# Autodesk Inventor assembly: nozzle
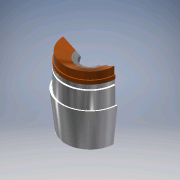
[picture p0: Inventor's stored thumbnail of the model, 180x180]
Saved by Autodesk Inventor 2017 (Build 210142000, 142)
## iProperties
Created: 2016-10-21
Part Number: nozzle
Document SubType Name: Assembly
Designer: cmflanne
Author: cmflanne
## Documents named in this file (7)
- C:\Users\cmflanne\Downloads\Intrepid\Nozzle\nozzle.iam
- C:\Users\cmflanne\Downloads\Intrepid\Nozzle\aluminum_carrier.ipt
- C:\Users\cmflanne\Downloads\Intrepid\Nozzle\aluminum_retainer.ipt
- C:\Users\cmflanne\Downloads\Intrepid\Nozzle\aluminum_skirt.ipt
- C:\Users\cmflanne\Downloads\Intrepid\Nozzle\graphite.ipt
- C:\Users\cmflanne\Downloads\Intrepid\Nozzle\phenolic_cap.ipt
- C:\Users\cmflanne\Downloads\Intrepid\Nozzle\phenolic_carrier.ipt
## Components (6 placed, 6 different names)
1. aluminum_carrier:1 — Mate:5, Mate:8, Mate:9, Mate:10
2. aluminum_retainer:1 — Mate:4, Mate:9
3. aluminum_skirt:1 — Mate:3, Mate:10
4. graphite:1 — Mate:1, Mate:2, Mate:3, Mate:4, Mate:5, Mate:6, Mate:7
5. phenolic_cap:1 — Mate:1, Mate:6, Mate:8
6. phenolic_carrier:1 — Mate:2, Mate:7
## Relationships (10: Mate 10)
- Mate:1: graphite:1 ↔ phenolic_cap:1
- Mate:2: graphite:1 ↔ phenolic_carrier:1
- Mate:3: aluminum_skirt:1 ↔ graphite:1
- Mate:4: aluminum_retainer:1 ↔ graphite:1
- Mate:5: aluminum_carrier:1 ↔ graphite:1
- Mate:6: graphite:1 ↔ phenolic_cap:1
- Mate:7: graphite:1 ↔ phenolic_carrier:1
- Mate:8: aluminum_carrier:1 ↔ phenolic_cap:1
- Mate:9: aluminum_carrier:1 ↔ aluminum_retainer:1
- Mate:10: aluminum_carrier:1 ↔ aluminum_skirt:1
